# Autodesk Inventor assembly: Train asembley
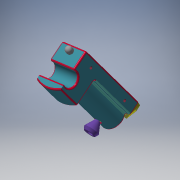
[picture p0: Inventor's stored thumbnail of the model, 180x180]
Saved by Autodesk Inventor 2017.1 (Build 211199000, 199)
## iProperties
Created: 2017-04-26
Part Number: Train asembley
Document SubType Name: Assembly
Designer: 196918
Author: 196918
## Documents named in this file (6)
- C:\Users\196918\Desktop\Train asembley.iam
- C:\Users\196918\Desktop\Cow pusher.ipt
- C:\Users\196918\Desktop\Train locomotive.ipt
- C:\Users\196918\Desktop\Train smoke stack.ipt
- C:\Users\196918\Desktop\Screw (train).ipt
- C:\Users\196918\Desktop\Washer (Train).ipt
## Components (5 placed, 5 different names)
1. Cow pusher:1 — Mate:1, Mate:2
2. Train locomotive:1 — Rigid:1, Mate:1, Mate:2, Rotational:1
3. Train smoke stack:1 — Rigid:1
4. Screw (train):1 — Rotational:2
5. Washer (Train):1 — Rotational:1, Rotational:2
## Relationships (5: Mate 2, RevoluteJoint 2, WeldJoint 1)
- Rigid:1 [WeldJoint]: Train locomotive:1 ↔ Train smoke stack:1
- Mate:1: Cow pusher:1 ↔ Train locomotive:1
- Mate:2: Cow pusher:1 ↔ Train locomotive:1
- Rotational:1 [RevoluteJoint]: Train locomotive:1 ↔ Washer (Train):1
- Rotational:2 [RevoluteJoint]: Screw (train):1 ↔ Washer (Train):1
